# Autodesk Inventor assembly: Solder Roll Support Assy
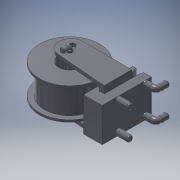
[picture p0: Inventor's stored thumbnail of the model, 180x180]
Saved by Autodesk Inventor 2016 (Build 200138000, 138)
## iProperties
Created: 2017-09-04
Part Number: Solder Roll Support Assy
Document SubType Name: Conjunto soldado
Designer: Zigunov
Weld Material: Aço macio soldado
Mass: 43548.6 g
Surface Area: 17698.1 cm^2
Volume: 5533.5 cm^3
Density: 7.87 g/cm^3
Author: Zigunov
## Documents named in this file (5)
- C:\Users\fzigu\Desktop\3D PRINTER\Designs\Lab Items\Solder Roll Support Assy.iam
- C:\Users\fzigu\Desktop\3D PRINTER\Designs\Lab Items\Solder Roll Support.ipt
- C:\Users\fzigu\Desktop\3D PRINTER\Designs\Lab Items\Solder Roll Support 2.ipt
- C:\Users\fzigu\Desktop\3D PRINTER\Designs\Lab Items\Solder Roll Support 3.ipt
- C:\Users\fzigu\Desktop\3D PRINTER\Designs\Lab Items\Solder Spool.ipt
## Components (4 placed, 4 different names)
1. Solder Roll Support:1 — Mate:1, Mate:2, Mate:3
2. Solder Roll Support 2:1 — Mate:1, Mate:2, Mate:3, Mate:4, Mate:5
3. Solder Roll Support 3:1 — Mate:4, Mate:5, Mate:6, Mate:7
4. Solder Spool:1 — Mate:6, Mate:7
## Relationships (7: Mate 7)
- Mate:1: Solder Roll Support:1 ↔ Solder Roll Support 2:1
- Mate:2 (3.85 mm): Solder Roll Support:1 ↔ Solder Roll Support 2:1
- Mate:3: Solder Roll Support:1 ↔ Solder Roll Support 2:1
- Mate:4: Solder Roll Support 2:1 ↔ Solder Roll Support 3:1
- Mate:5: Solder Roll Support 2:1 ↔ Solder Roll Support 3:1
- Mate:6: Solder Roll Support 3:1 ↔ Solder Spool:1
- Mate:7: Solder Roll Support 3:1 ↔ Solder Spool:1
